# Autodesk Inventor assembly: thick screw motor
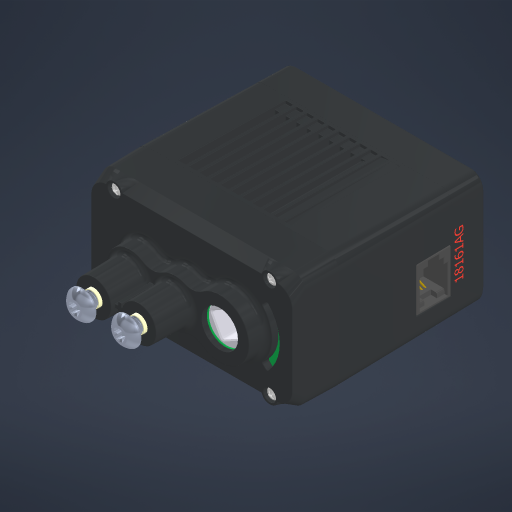
[picture p0: Inventor's stored thumbnail of the model, 512x512]
Saved by Autodesk Inventor 2024 (Build 280153000, 153)
## iProperties
Created: 2024-01-05
Part Number: thick screw motor
Document SubType Name: Assembly
Designer: macbook
Author: macbook
## Documents named in this file (4)
- \\Mac\Home\Desktop\code\1599V-VRC\Cad\Assembly\thick screw motor.iam
- \\Mac\Home\Desktop\code\1599V-VRC\Cad\Electronics\V5 Motor.ipt
- \\Mac\Home\Desktop\code\1599V-VRC\Cad\Structure\Hardware\Screw Steel - Star\SScrew Star Threaded .500.ipt
- \\Mac\Home\Desktop\code\1599V-VRC\Cad\Structure\Hardware\Screw Steel - Star.ipt
## Components (3 placed, 2 different names)
1. V5 Motor:1 — Insert:1, Insert:2
2. SScrew Star Threaded .500:1 — Insert:1
3. SScrew Star Threaded .500:2 — Insert:2
## Relationships (2: Insert 2)
- Insert:1 (3.175 mm): V5 Motor:1 ↔ SScrew Star Threaded .500:1
- Insert:2 (3.175 mm): V5 Motor:1 ↔ SScrew Star Threaded .500:2
